# Autodesk Inventor assembly: Assembly2
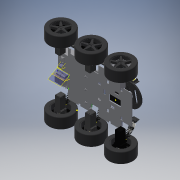
[picture p0: Inventor's stored thumbnail of the model, 180x180]
Saved by Autodesk Inventor 2016 (Build 200138000, 138)
## iProperties
Created: 2015-06-07
Part Number: Assembly2
Document SubType Name: Assembly
Designer: Jufo
Author: Jufo
## Documents named in this file (26)
- C:\Users\Juraj\Documents\GitHub\Robot6x6\Terrenny robot CAD\robot.iam
- C:\Users\Juraj\Documents\GitHub\Robot6x6\Terrenny robot CAD\spodok2.ipt
- C:\Users\Juraj\Documents\GitHub\Robot6x6\Terrenny robot CAD\spodok1.ipt
- C:\Users\Juraj\Documents\GitHub\Robot6x6\Terrenny robot CAD\Kinect\kinect assembly.iam
- C:\Users\Juraj\Documents\GitHub\Robot6x6\Terrenny robot CAD\bateria.ipt
- C:\Users\Juraj\Documents\GitHub\Robot6x6\Terrenny robot CAD\M3x6.ipt
- C:\Users\Juraj\Documents\GitHub\Robot6x6\Terrenny robot CAD\raspberry-pi-2-model-b-3d-cad-assembly-model-2.snapshot.18\Imported Components\RaspberryPi2 STEP214\RaspberryPi2 STEP214.iam
- C:\Users\Juraj\Documents\GitHub\Robot6x6\Terrenny robot CAD\stred2.ipt
- C:\Users\Juraj\Documents\GitHub\Robot6x6\Terrenny robot CAD\vrch1.ipt
- C:\Users\Juraj\Documents\GitHub\Robot6x6\Terrenny robot CAD\vrch2.ipt
- C:\Users\Juraj\Documents\GitHub\Robot6x6\Terrenny robot CAD\mg996r-servo.snapshot.1\MG996R\Imported Components\MG996R\MG996R.iam
- C:\Users\Juraj\Documents\GitHub\Robot6x6\Terrenny robot CAD\kinectUchyt.ipt
- C:\Users\Juraj\Documents\GitHub\Robot6x6\Terrenny robot CAD\arduino-l298n-1.snapshot.1\L298N.ipt
- C:\Users\Juraj\Documents\GitHub\Robot6x6\Terrenny robot CAD\router.ipt
- C:\Users\Juraj\Documents\GitHub\Robot6x6\Terrenny robot CAD\stred1.ipt
- C:\Users\Juraj\Documents\GitHub\Robot6x6\Terrenny robot CAD\relay_module.ipt
- C:\Users\Juraj\Documents\GitHub\Robot6x6\Terrenny robot CAD\DC menic.ipt
- C:\Users\Juraj\Documents\GitHub\Robot6x6\Terrenny robot CAD\wifi-antenna-1.snapshot.1\Imported Components\Antenna hub\Antenna hub.ipt
- C:\Users\Juraj\Documents\GitHub\Robot6x6\Terrenny robot CAD\wifi-antenna-1.snapshot.1\Imported Components\Antennae\Antennae.ipt
- C:\Users\Juraj\Documents\GitHub\Robot6x6\Terrenny robot CAD\tlacitko.ipt
- C:\Users\Juraj\Documents\GitHub\Robot6x6\Terrenny robot CAD\rj45.ipt
- C:\Users\Juraj\Documents\GitHub\Robot6x6\Terrenny robot CAD\GPS sensor.ipt
- C:\Users\Juraj\Documents\GitHub\Robot6x6\Terrenny robot CAD\ACS712(prudovy snimac).ipt
- C:\Users\Juraj\Documents\GitHub\Robot6x6\Terrenny robot CAD\accelerometer.ipt
- C:\Users\Juraj\Documents\GitHub\Robot6x6\Terrenny robot CAD\arduino-pro-mini-1.snapshot.4\Arduino Pro Mini\Arduino_pro_mini.ipt
- C:\Users\Juraj\Documents\GitHub\Robot6x6\Terrenny robot CAD\motormodul.iam
## Components (47 placed, 25 different names)
1. accelerometer:1 — Mate:56
2. rj45:1 — Mate:57, Mate:58, Mate:59
3. GPS sensor:1 — Mate:60
4. tlacitko:3 — Insert:96
5. tlacitko:2 — Insert:95
6. tlacitko:1 — Insert:97
7. Antenna hub:1 — Insert:86, Insert:87
8. Antenna hub:2 — Insert:85, Insert:88
9. Antennae:2 — Insert:85
10. Antennae:1 — Insert:86
11. vrch1:1 — Insert:65, Insert:66, Insert:69, Insert:70, Mate:56
12. vrch2:1 — Insert:67, Insert:68, Insert:87, Insert:88, Mate:57, Mate:58, Mate:59, Mate:60, Insert:95, Insert:96, Insert:97
13. kinect assembly:1 [sub-assembly] — Insert:72
14. relay_module:1 — Insert:98, Insert:99
15. DC menic:2 — Insert:111
16. DC menic:1 — Insert:110
17. ACS712(prudovy snimac):1 — Mate:54, Mate:55
18. RaspberryPi2 STEP214:1 [sub-assembly] — Insert:102, Insert:103
19. router:1 — Mate:38
20. L298N:1 — Insert:115, Insert:116
21. L298N:2 — Insert:113, Insert:114
22. L298N:3 — Insert:117, Insert:118
23. medzicast_zadna — Insert:75, Insert:76, Mate:54, Insert:98, Insert:99, Insert:102, Insert:103
24. medzicast_predna — Mate:38, Insert:73, Insert:74, Mate:63, Mate:65, Mate:74, Mate:75, Insert:110, Insert:111, Insert:112, Insert:113, Insert:114, Insert:115, Insert:116, Insert:117, Insert:118
25. spodok_predny — Insert:1, Insert:10, Insert:65, Insert:66, Insert:73, Insert:74, Insert:122, Insert:123, Insert:124, Insert:125, Insert:126, Insert:127, Insert:134, Insert:135, Insert:136, Insert:137, Insert:138, Insert:139
26. spodok_zadny — Insert:1, Insert:10, Insert:56, Insert:57, Insert:58, Insert:59, Insert:60, Insert:61, Insert:67, Insert:68, Insert:75, Insert:76, Mate:41, Mate:42, Mate:43, Mate:44, Mate:45, Mate:46, Insert:119, Insert:120, Insert:121, Insert:128, Insert:129, Insert:130
27. bateria:1 — Mate:41, Mate:44, Mate:45, Mate:55
28. bateria:2 — Mate:42, Mate:43, Mate:46
29. DC menic:3 — Insert:112
30. Arduino_pro_mini:3 — Mate:65
31. Arduino_pro_mini:2 — Mate:74
32. Arduino_pro_mini:1 — Mate:63, Mate:75
33. motormodul:1 [sub-assembly] — Insert:122, Insert:123, Insert:124
34. motormodul:2 [sub-assembly] — Insert:125, Insert:126, Insert:127
35. motormodul:3 [sub-assembly] — Insert:134, Insert:135, Insert:136
36. motormodul:4 [sub-assembly] — Insert:137, Insert:138, Insert:139
37. motormodul:5 [sub-assembly] — Insert:119, Insert:120, Insert:121
38. motormodul:6 [sub-assembly] — Insert:128, Insert:129, Insert:130
39. M3x6:1 — Insert:56
40. M3x6:2 — Insert:59
41. M3x6:3 — Insert:60
42. M3x6:4 — Insert:57
43. M3x6:5 — Insert:58
44. M3x6:8
45. M3x6:9 — Insert:61
46. MG996R:1 [sub-assembly] — Insert:69, Insert:70, Insert:71
47. kinectUchyt:1 — Insert:71, Insert:72
## Relationships (76: Insert 58, Mate 18)
- Insert:1: spodok_predny ↔ spodok_zadny
- Insert:10: spodok_predny ↔ spodok_zadny
- Insert:56 (-6 mm): spodok_zadny ↔ M3x6:1
- Insert:57 (-6 mm): spodok_zadny ↔ M3x6:4
- Insert:58 (-6 mm): spodok_zadny ↔ M3x6:5
- Insert:59 (-6 mm): spodok_zadny ↔ M3x6:2
- Insert:60 (-6 mm): spodok_zadny ↔ M3x6:3
- Insert:61 (-6 mm): spodok_zadny ↔ M3x6:9
- Insert:65: vrch1:1 ↔ spodok_predny
- Insert:66: vrch1:1 ↔ spodok_predny
- Insert:67: vrch2:1 ↔ spodok_zadny
- Insert:68: vrch2:1 ↔ spodok_zadny
- Insert:69: vrch1:1 ↔ MG996R:1
- Insert:70: vrch1:1 ↔ MG996R:1
- Insert:71: MG996R:1 ↔ kinectUchyt:1
- Mate:38: router:1 ↔ medzicast_predna
- Insert:72: kinect assembly:1 ↔ kinectUchyt:1
- Insert:73: medzicast_predna ↔ spodok_predny
- Insert:74: medzicast_predna ↔ spodok_predny
- Insert:75: medzicast_zadna ↔ spodok_zadny
- Insert:76: medzicast_zadna ↔ spodok_zadny
- Mate:41: spodok_zadny ↔ bateria:1
- Mate:42: spodok_zadny ↔ bateria:2
- Mate:43 (1 mm): spodok_zadny ↔ bateria:2
- Mate:44 (1 mm): spodok_zadny ↔ bateria:1
- Mate:45 (1 mm): spodok_zadny ↔ bateria:1
- Mate:46: spodok_zadny ↔ bateria:2
- Insert:85: Antenna hub:2 ↔ Antennae:2
- Insert:86: Antenna hub:1 ↔ Antennae:1
- Insert:87: Antenna hub:1 ↔ vrch2:1
- Insert:88: Antenna hub:2 ↔ vrch2:1
- Mate:54: ACS712(prudovy snimac):1 ↔ medzicast_zadna
- Mate:55 (20 mm): ACS712(prudovy snimac):1 ↔ bateria:1
- Mate:56: accelerometer:1 ↔ vrch1:1
- Mate:57 (-4 mm): rj45:1 ↔ vrch2:1
- Mate:58 (0.5 mm): rj45:1 ↔ vrch2:1
- Mate:59 (0.5 mm): rj45:1 ↔ vrch2:1
- Mate:60 (0.3 mm): GPS sensor:1 ↔ vrch2:1
- Insert:95: tlacitko:2 ↔ vrch2:1
- Insert:96: tlacitko:3 ↔ vrch2:1
- Insert:97: tlacitko:1 ↔ vrch2:1
- Insert:98: relay_module:1 ↔ medzicast_zadna
- Insert:99: relay_module:1 ↔ medzicast_zadna
- Insert:102: RaspberryPi2 STEP214:1 ↔ medzicast_zadna
- Insert:103: RaspberryPi2 STEP214:1 ↔ medzicast_zadna
- Mate:63: medzicast_predna ↔ Arduino_pro_mini:1
- Mate:65: medzicast_predna ↔ Arduino_pro_mini:3
- Mate:74: medzicast_predna ↔ Arduino_pro_mini:2
- Mate:75 (55 mm): medzicast_predna ↔ Arduino_pro_mini:1
- Insert:110: DC menic:1 ↔ medzicast_predna
- Insert:111: DC menic:2 ↔ medzicast_predna
- Insert:112: medzicast_predna ↔ DC menic:3
- Insert:113: L298N:2 ↔ medzicast_predna
- Insert:114: L298N:2 ↔ medzicast_predna
- Insert:115: L298N:1 ↔ medzicast_predna
- Insert:116: L298N:1 ↔ medzicast_predna
- Insert:117: L298N:3 ↔ medzicast_predna
- Insert:118: L298N:3 ↔ medzicast_predna
- Insert:119: spodok_zadny ↔ motormodul:5
- Insert:120: spodok_zadny ↔ motormodul:5
- Insert:121 (0.5 mm): spodok_zadny ↔ motormodul:5
- Insert:122: spodok_predny ↔ motormodul:1
- Insert:123: spodok_predny ↔ motormodul:1
- Insert:124 (0.5 mm): spodok_predny ↔ motormodul:1
- Insert:125: spodok_predny ↔ motormodul:2
- Insert:126: spodok_predny ↔ motormodul:2
- Insert:127 (0.5 mm): spodok_predny ↔ motormodul:2
- Insert:128: spodok_zadny ↔ motormodul:6
- Insert:129: spodok_zadny ↔ motormodul:6
- Insert:130 (0.5 mm): spodok_zadny ↔ motormodul:6
- Insert:134: spodok_predny ↔ motormodul:3
- Insert:135: spodok_predny ↔ motormodul:3
- Insert:136 (0.5 mm): spodok_predny ↔ motormodul:3
- Insert:137: spodok_predny ↔ motormodul:4
- Insert:138: spodok_predny ↔ motormodul:4
- Insert:139 (0.5 mm): spodok_predny ↔ motormodul:4
